# Autodesk Inventor assembly: Montagem
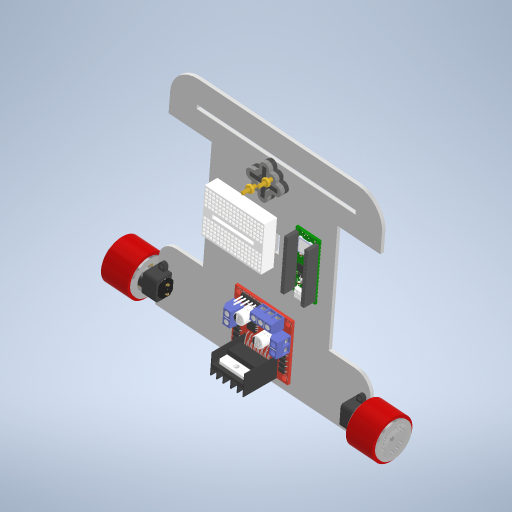
[picture p0: Inventor's stored thumbnail of the model, 512x512]
Saved by Autodesk Inventor 2024.2 (Build 282272000, 272)
## iProperties
Created: 2024-04-09
Part Number: Montagem
Document SubType Name: Assembly
Designer: Documentos
Author: Documentos
## Documents named in this file (7)
- C:\Users\Documentos\Documents\Inventor\Protótipo - Segue Faixa\Montagem.iam
- C:\Users\Documentos\Documents\Inventor\Protótipo - Segue Faixa\Peça1.ipt
- C:\Users\Documentos\Documents\Inventor\Protótipo - Segue Faixa\Ponte L298H\Ponte L298H.ipt
- C:\Users\Documentos\Documents\Inventor\Protótipo - Segue Faixa\Esfera deslizante\Esfera deslizante.ipt
- C:\Users\Documentos\Documents\Inventor\Protótipo - Segue Faixa\Motor\GearMotor\Motor - Completo.iam
- C:\Users\Documentos\Documents\Inventor\Protótipo - Segue Faixa\Mini Protoboard\MINIPROTOBOARD\MINIPROTOBOARD.ipt
- C:\Users\Documentos\Documents\Inventor\Protótipo - Segue Faixa\Arduino Nano\ArduinoNanoESP32\ArduinoNanoESP32.ipt
## Components (7 placed, 6 different names)
1. Ponte L298H:1 — Coincidente:15, Coincidente:16, Coincidente:22
2. Peça1:1 — Coincidente:1, Coincidente:2, Coincidente:3, Coincidente:4, Coincidente:5, Coincidente:6, Coincidente:7, Coincidente:8, Coincidente:9, Coincidente:10, Coincidente:11, Coincidente:12, Coincidente:13, Coincidente:14, Coincidente:15, Coincidente:16, Coincidente:18, Coincidente:19, Coincidente:20, Coincidente:21, Coincidente:22
3. Esfera deslizante:1 — Coincidente:19, Coincidente:20, Coincidente:21
4. GearMotor:1 [sub-assembly] — Coincidente:12, Coincidente:13, Coincidente:14
5. GearMotor:2 [sub-assembly] — Coincidente:8, Coincidente:9, Coincidente:10, Coincidente:11
6. MINIPROTOBOARD:1 — Coincidente:1, Coincidente:2, Coincidente:18
7. ArduinoNanoESP32:1 — Coincidente:3, Coincidente:4, Coincidente:5, Coincidente:6, Coincidente:7
## Relationships (21: Mate 21)
- Coincidente:1 [Mate]: Peça1:1 ↔ MINIPROTOBOARD:1
- Coincidente:2 [Mate]: Peça1:1 ↔ MINIPROTOBOARD:1
- Coincidente:3 [Mate]: Peça1:1 ↔ ArduinoNanoESP32:1
- Coincidente:4 [Mate]: Peça1:1 ↔ ArduinoNanoESP32:1
- Coincidente:5 [Mate]: Peça1:1 ↔ ArduinoNanoESP32:1
- Coincidente:6 [Mate]: Peça1:1 ↔ ArduinoNanoESP32:1
- Coincidente:7 [Mate]: Peça1:1 ↔ ArduinoNanoESP32:1
- Coincidente:8 [Mate]: Peça1:1 ↔ GearMotor:2
- Coincidente:9 [Mate]: Peça1:1 ↔ GearMotor:2
- Coincidente:10 [Mate]: Peça1:1 ↔ GearMotor:2
- Coincidente:11 [Mate]: Peça1:1 ↔ GearMotor:2
- Coincidente:12 [Mate]: Peça1:1 ↔ GearMotor:1
- Coincidente:13 [Mate]: Peça1:1 ↔ GearMotor:1
- Coincidente:14 [Mate]: Peça1:1 ↔ GearMotor:1
- Coincidente:15 [Mate]: Ponte L298H:1 ↔ Peça1:1
- Coincidente:16 [Mate]: Ponte L298H:1 ↔ Peça1:1
- Coincidente:18 [Mate] (-10.441 mm): Peça1:1 ↔ MINIPROTOBOARD:1
- Coincidente:19 [Mate]: Peça1:1 ↔ Esfera deslizante:1
- Coincidente:20 [Mate]: Peça1:1 ↔ Esfera deslizante:1
- Coincidente:21 [Mate]: Peça1:1 ↔ Esfera deslizante:1
- Coincidente:22 [Mate] (0.001 mm): Ponte L298H:1 ↔ Peça1:1
